# Autodesk Inventor assembly: 1000_Full_Assembly_MPSv2_v2
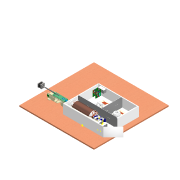
[picture p0: Inventor's stored thumbnail of the model, 180x180]
Saved by Autodesk Inventor 2021 (Build 250183000, 183)
## iProperties
Created: 2020-11-18
Part Number: 1000_Full_Assembly_MPSv2_v2
Document SubType Name: Assembly
Designer: Admin
Author: Admin
## Documents named in this file (8)
- C:\Users\Eli\Documents\GitHub\MPS\Inventor Parts\MPSV2\1xxx Assemblies\1000_Full_Assembly_MPSv2_v2.iam
- C:\Users\Eli\Documents\GitHub\MPS\Inventor Parts\MPSV2\1xxx Assemblies\11xx_PCB_Assemblies\110x_Drive_Amplifier_Assemblies\1100_Drive_Amplifier_Heatsink_MPSv2_v1.iam
- C:\Users\Eli\Documents\GitHub\MPS\Inventor Parts\MPSV2\1xxx Assemblies\1000_Coil_Positioning_Assembly_MPSv2_v4.iam
- C:\Users\Eli\Documents\GitHub\MPS\Inventor Parts\MPSV2\4xxx PCB and Filters\41xx Tx Filter\413x Tx Filter Layout\8100_Tx_Filter_Stage2_Layout_v2.iam
- C:\Users\Eli\Documents\GitHub\MPS\Inventor Parts\MPSV2\4xxx PCB and Filters\41xx Tx Filter\413x Tx Filter Layout\8100_Tx_Filter_Stage1_Layout_v2.iam
- C:\Users\Eli\Documents\GitHub\MPS\Inventor Parts\MPSV2\5xxx Enclosures\50xx Aluminum Chasis\5010_1444-17154_[DigiKey]_Aluminum_Chasis_Modification_MPSv2_V1.iam
- C:\Users\Eli\Documents\GitHub\MPS\Inventor Parts\MPSV2\5xxx Enclosures\5100_Base_Board_MPSv2_v1.ipt
- C:\Users\Eli\Documents\GitHub\MPS\Inventor Parts\MPSV2\6xxx_Sample Assembly\6000_Sample Assembly_V3.iam
## Components (8 placed, 7 different names)
1. 5010_1444-17154_[DigiKey]_Aluminum_Chasis_Modification_MPSv2_V1:1 [sub-assembly] — Mate:5, Mate:6, Mate:9, Mate:10, Angle:1, Mate:12, Mate:14, Angle:2, Mate:15, Angle:3, Mate:16, Angle:4, Mate:17, Flush:2, Flush:3
2. 1000_Coil_Positioning_Assembly_MPSv2_v4:1 [sub-assembly] — Mate:5, Mate:6, Mate:12, Mate:19
3. 1100_Drive_Amplifier_Heatsink_MPSv2_v1:1 [sub-assembly] — Mate:10, Mate:11, Flush:1
4. 1100_Drive_Amplifier_Heatsink_MPSv2_v1:2 [sub-assembly] — Mate:9, Mate:11, Flush:1, Angle:1
5. 8100_Tx_Filter_Stage2_Layout_v2:1 [sub-assembly] — Mate:15, Angle:3
6. 8100_Tx_Filter_Stage1_Layout_v2:1 [sub-assembly] — Mate:14, Angle:2
7. 5100_Base_Board_MPSv2_v1:1 — Mate:16, Angle:4, Mate:18, Flush:2, Flush:3
8. 6000_Sample Assembly_V3:1 [sub-assembly] — Mate:17, Mate:18, Mate:19
## Relationships (19: Mate 12, Angle 4, Flush 3)
- Mate:5: 5010_1444-17154_[DigiKey]_Aluminum_Chasis_Modification_MPSv2_V1:1 ↔ 1000_Coil_Positioning_Assembly_MPSv2_v4:1
- Mate:6: 5010_1444-17154_[DigiKey]_Aluminum_Chasis_Modification_MPSv2_V1:1 ↔ 1000_Coil_Positioning_Assembly_MPSv2_v4:1
- Mate:9: 5010_1444-17154_[DigiKey]_Aluminum_Chasis_Modification_MPSv2_V1:1 ↔ 1100_Drive_Amplifier_Heatsink_MPSv2_v1:2
- Mate:10: 5010_1444-17154_[DigiKey]_Aluminum_Chasis_Modification_MPSv2_V1:1 ↔ 1100_Drive_Amplifier_Heatsink_MPSv2_v1:1
- Mate:11: 1100_Drive_Amplifier_Heatsink_MPSv2_v1:1 ↔ 1100_Drive_Amplifier_Heatsink_MPSv2_v1:2
- Flush:1: 1100_Drive_Amplifier_Heatsink_MPSv2_v1:1 ↔ 1100_Drive_Amplifier_Heatsink_MPSv2_v1:2
- Angle:1 (180 deg): 5010_1444-17154_[DigiKey]_Aluminum_Chasis_Modification_MPSv2_V1:1 ↔ 1100_Drive_Amplifier_Heatsink_MPSv2_v1:2
- Mate:12: 5010_1444-17154_[DigiKey]_Aluminum_Chasis_Modification_MPSv2_V1:1 ↔ 1000_Coil_Positioning_Assembly_MPSv2_v4:1
- Mate:14: 5010_1444-17154_[DigiKey]_Aluminum_Chasis_Modification_MPSv2_V1:1 ↔ 8100_Tx_Filter_Stage1_Layout_v2:1
- Angle:2 (90 deg): 5010_1444-17154_[DigiKey]_Aluminum_Chasis_Modification_MPSv2_V1:1 ↔ 8100_Tx_Filter_Stage1_Layout_v2:1
- Mate:15: 5010_1444-17154_[DigiKey]_Aluminum_Chasis_Modification_MPSv2_V1:1 ↔ 8100_Tx_Filter_Stage2_Layout_v2:1
- Angle:3 (0 deg): 5010_1444-17154_[DigiKey]_Aluminum_Chasis_Modification_MPSv2_V1:1 ↔ 8100_Tx_Filter_Stage2_Layout_v2:1
- Mate:16: 5010_1444-17154_[DigiKey]_Aluminum_Chasis_Modification_MPSv2_V1:1 ↔ 5100_Base_Board_MPSv2_v1:1
- Angle:4 (0 deg): 5010_1444-17154_[DigiKey]_Aluminum_Chasis_Modification_MPSv2_V1:1 ↔ 5100_Base_Board_MPSv2_v1:1
- Mate:17: 5010_1444-17154_[DigiKey]_Aluminum_Chasis_Modification_MPSv2_V1:1 ↔ 6000_Sample Assembly_V3:1
- Mate:18: 5100_Base_Board_MPSv2_v1:1 ↔ 6000_Sample Assembly_V3:1
- Mate:19: 1000_Coil_Positioning_Assembly_MPSv2_v4:1 ↔ 6000_Sample Assembly_V3:1
- Flush:2 (50 mm): 5010_1444-17154_[DigiKey]_Aluminum_Chasis_Modification_MPSv2_V1:1 ↔ 5100_Base_Board_MPSv2_v1:1
- Flush:3 (150 mm): 5010_1444-17154_[DigiKey]_Aluminum_Chasis_Modification_MPSv2_V1:1 ↔ 5100_Base_Board_MPSv2_v1:1
